# Autodesk Inventor assembly: DriveChain2
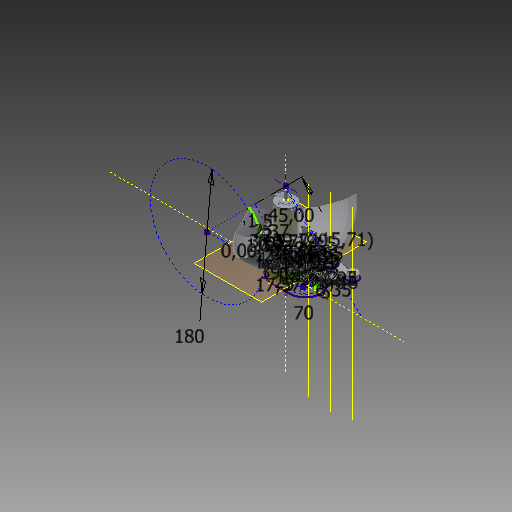
[picture p0: Inventor's stored thumbnail of the model, 512x512]
Saved by Autodesk Inventor 2018.3 (Build 223284000, 284)
## iProperties
Created: 2018-07-27
Part Number: DriveChain2
Material: Generisch
Document SubType Name: Assembly
Designer: JochenAlt
Author: JochenAlt
## Documents named in this file (10)
- D:\Projects\FlowerPot\CAD\DriveChain.iam
- D:\Projects\FlowerPot\CAD\DriveChainEnclosure2.ipt
- D:\Projects\FlowerPot\CAD\Motor.iam
- C:\Users\JochenAlt\Documents\Inventor\Content Center Files\R2018\de-DE\DIN BEARING(1)\DIN 625 SKF - SKF 623.ipt
- D:\Projects\FlowerPot\CAD\HarmonicDrive-Axis.ipt
- D:\Projects\FlowerPot\CAD\BushOmniWheel.ipt
- D:\Projects\FlowerPot\CAD\OmniWheel-66mm.ipt
- D:\Projects\FlowerPot\CAD\Mounting Hub.ipt
- D:\Projects\FlowerPot\CAD\Encoder\Avago Encoder.iam
- D:\Projects\FlowerPot\CAD\Beltdrive\BeltDriveConstruction.iam
## Components (11 placed, 9 different names)
1. DriveChainEnclosure:1 — Passend:7, Passend:8, Passend:9, Passend:10, Passend:18, Passend:27
2. Motor:1 [sub-assembly] — Passend:31, Passend:33
3. DIN 625 SKF SKF 623:1 — Passend:7
4. HarmonicDrive-Axis:1 — Passend:8, Passend:11, Passend:13, Drehung:4, Passend:15, Passend:17, Passend:26, Drehung:5, Passend:34
5. DIN 625 SKF SKF 623:2 — Passend:9, Passend:10, Passend:12
6. BushOmniWheel:1 — Passend:11, Passend:12, Passend:14
7. OmniWheel:1 — Passend:15, Passend:16, Drehung:6
8. Mounting Hub:1 — Passend:13, Drehung:4, Passend:14, Passend:16, Drehung:6
9. Avago Encoder:1 [sub-assembly] — Passend:17, Passend:18
10. BeltDriveConstruction:1 [sub-assembly] — Passend:31, Passend:32, Passend:33, Passend:34, Passend:35
11. Mounting Hub:3 — Passend:26, Passend:27, Drehung:5, Passend:35
## Relationships (22: Mate 19, RelateRotation 3)
- Passend:7 [Mate]: DriveChainEnclosure:1 ↔ DIN 625 SKF SKF 623:1
- Passend:8 [Mate]: DriveChainEnclosure:1 ↔ HarmonicDrive-Axis:1
- Passend:9 [Mate]: DriveChainEnclosure:1 ↔ DIN 625 SKF SKF 623:2
- Passend:10 [Mate]: DriveChainEnclosure:1 ↔ DIN 625 SKF SKF 623:2
- Passend:11 [Mate]: HarmonicDrive-Axis:1 ↔ BushOmniWheel:1
- Passend:12 [Mate]: DIN 625 SKF SKF 623:2 ↔ BushOmniWheel:1
- Passend:13 [Mate]: HarmonicDrive-Axis:1 ↔ Mounting Hub:1
- Drehung:4 [RelateRotation] (-1 ul): HarmonicDrive-Axis:1 ↔ Mounting Hub:1
- Passend:14 [Mate]: BushOmniWheel:1 ↔ Mounting Hub:1
- Passend:15 [Mate]: HarmonicDrive-Axis:1 ↔ OmniWheel:1
- Passend:16 [Mate]: OmniWheel:1 ↔ Mounting Hub:1
- Passend:17 [Mate]: HarmonicDrive-Axis:1 ↔ Avago Encoder:1
- Passend:18 [Mate]: DriveChainEnclosure:1 ↔ Avago Encoder:1
- Passend:26 [Mate]: HarmonicDrive-Axis:1 ↔ Mounting Hub:3
- Passend:27 [Mate] (1 mm): DriveChainEnclosure:1 ↔ Mounting Hub:3
- Drehung:5 [RelateRotation] (1 ul): HarmonicDrive-Axis:1 ↔ Mounting Hub:3
- Drehung:6 [RelateRotation] (1 ul): OmniWheel:1 ↔ Mounting Hub:1
- Passend:31 [Mate]: Motor:1 ↔ BeltDriveConstruction:1
- Passend:32 [Mate]: BeltDriveConstruction:1
- Passend:33 [Mate] (17.5 mm): Motor:1 ↔ BeltDriveConstruction:1
- Passend:34 [Mate]: HarmonicDrive-Axis:1 ↔ BeltDriveConstruction:1
- Passend:35 [Mate]: BeltDriveConstruction:1 ↔ Mounting Hub:3
